# Autodesk Inventor assembly: GRUÚA
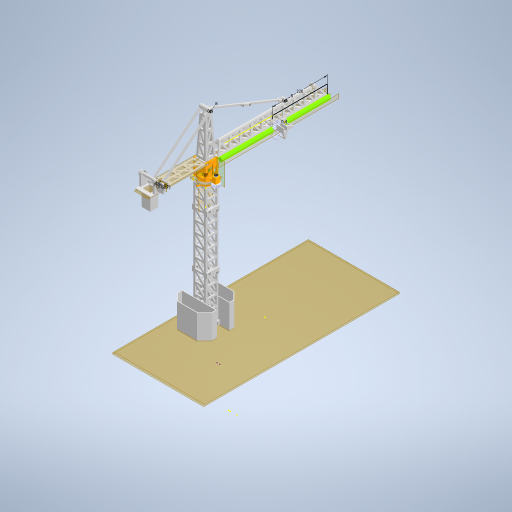
[picture p0: Inventor's stored thumbnail of the model, 512x512]
Saved by Autodesk Inventor 2023 (Build 270158000, 158)
## iProperties
Created: 2024-07-07
Part Number: GRUÚA
Document SubType Name: Assembly
Designer: Usuario
Author: Usuario
## Documents named in this file (16)
- C:\Users\Usuario\Desktop\GRUA\GRUÚA.iam
- C:\Users\Usuario\Desktop\GRUA\ALOJAMIENTO MOTOR.ipt
- C:\Users\Usuario\Desktop\GRUA\CARRIL 1.ipt
- C:\Users\Usuario\Downloads\CABLE 3_MIR.ipt
- C:\Users\Usuario\Downloads\CABLE 3_2_MIR.ipt
- C:\Users\Usuario\Downloads\CABLE 3_MIR1.ipt
- C:\Users\Usuario\Downloads\CABLE 3_2_MIR1.ipt
- C:\Users\Usuario\Downloads\CABLE 3_MIR2.ipt
- C:\Users\Usuario\Downloads\CABLE 3_2_MIR2.ipt
- C:\Users\Usuario\Desktop\GRUA\GRUA INF.ipt
- C:\Users\Usuario\Desktop\GRUA\GRÚA SUP.ipt
- C:\Users\Usuario\Documents\Inventor\Content Center Files\R2023\es-ES\ANSI B18.3.4M(1)\ANSI B18.3.4M - M4 x 0.7 x 12(2).ipt
- C:\Users\Usuario\Desktop\GRUA\Pieza26.ipt
- C:\Users\Usuario\Desktop\GRUA\Carril 1 ipt.ipt
- C:\Users\Usuario\Desktop\GRUA\Union engranaje.ipt
- C:\Users\Usuario\Desktop\GRUA\CARRIL Y RUEDAS DEFINITIVO.ipt
## Components (34 placed, 15 different names)
1. CABLE 3_MIR:1
2. CABLE 3_2_MIR:1
3. CABLE 3_MIR1:1
4. CABLE 3_2_MIR1:1
5. CABLE 3_MIR2:1
6. CABLE 3_2_MIR2:1
7. GRUA INF:1 — De rotación:6, De rotación:7, De rotación:10, De rotación:11, De rotación:12, De rotación:13, De rotación:17, De rotación:18, De rotación:19, De rotación:20, De rotación:21, De rotación:22
8. ALOJAMIENTO MOTOR:1 — De rotación:3, De rotación:26
9. GRÚA SUP:1 — De rotación:3, De rotación:5, De rotación:14, De rotación:15, De rotación:16, De rotación:23, De rotación:24, De rotación:25, Rígido:1, Coincidencia:1, Cilíndrica:1
10. CARRIL 1:1 — De rotación:5
11. Tornillo brochado de cabeza de botón hexagonal hueca - Métrico M4 x 0.7 x 12:1 — De rotación:6
12. Tornillo brochado de cabeza de botón hexagonal hueca - Métrico M4 x 0.7 x 12:2 — De rotación:12
13. Tornillo brochado de cabeza de botón hexagonal hueca - Métrico M4 x 0.7 x 12:3
14. Tornillo brochado de cabeza de botón hexagonal hueca - Métrico M4 x 0.7 x 12:4 — De rotación:10
15. Tornillo brochado de cabeza de botón hexagonal hueca - Métrico M4 x 0.7 x 12:5 — De rotación:11
16. Tornillo brochado de cabeza de botón hexagonal hueca - Métrico M4 x 0.7 x 12:6 — De rotación:13
17. Tornillo brochado de cabeza de botón hexagonal hueca - Métrico M4 x 0.7 x 12:7 — De rotación:7
18. Tornillo brochado de cabeza de botón hexagonal hueca - Métrico M4 x 0.7 x 12:8
19. Tornillo brochado de cabeza de botón hexagonal hueca - Métrico M4 x 0.7 x 12:9 — De rotación:14
20. Tornillo brochado de cabeza de botón hexagonal hueca - Métrico M4 x 0.7 x 12:10 — De rotación:16
21. Tornillo brochado de cabeza de botón hexagonal hueca - Métrico M4 x 0.7 x 12:11 — De rotación:15
22. Tornillo brochado de cabeza de botón hexagonal hueca - Métrico M4 x 0.7 x 12:12 — De rotación:17
23. Tornillo brochado de cabeza de botón hexagonal hueca - Métrico M4 x 0.7 x 12:13 — De rotación:18
24. Tornillo brochado de cabeza de botón hexagonal hueca - Métrico M4 x 0.7 x 12:14 — De rotación:19
25. Tornillo brochado de cabeza de botón hexagonal hueca - Métrico M4 x 0.7 x 12:15 — De rotación:20
26. Tornillo brochado de cabeza de botón hexagonal hueca - Métrico M4 x 0.7 x 12:16 — De rotación:21
27. Tornillo brochado de cabeza de botón hexagonal hueca - Métrico M4 x 0.7 x 12:17 — De rotación:22
28. Tornillo brochado de cabeza de botón hexagonal hueca - Métrico M4 x 0.7 x 12:18 — De rotación:23
29. Tornillo brochado de cabeza de botón hexagonal hueca - Métrico M4 x 0.7 x 12:19 — De rotación:24
30. Tornillo brochado de cabeza de botón hexagonal hueca - Métrico M4 x 0.7 x 12:20 — De rotación:25
31. Pieza26:1 — Rígido:1
32. Carril 1 ipt:1 — Coincidencia:1, Cilíndrica:1, Rígido:2
33. Union engranaje:1 — De rotación:26
34. CARRIL Y RUEDAS DEFINITIVO:1 — Rígido:2
## Relationships (25: RevoluteJoint 21, WeldJoint 2, Mate 1, CylindricalJoint 1)
- De rotación:3 [RevoluteJoint]: ALOJAMIENTO MOTOR:1 ↔ GRÚA SUP:1
- De rotación:5 [RevoluteJoint]: GRÚA SUP:1 ↔ CARRIL 1:1
- De rotación:6 [RevoluteJoint]: GRUA INF:1 ↔ Tornillo brochado de cabeza de botón hexagonal hueca - Métrico M4 x 0.7 x 12:1
- De rotación:7 [RevoluteJoint]: GRUA INF:1 ↔ Tornillo brochado de cabeza de botón hexagonal hueca - Métrico M4 x 0.7 x 12:7
- De rotación:10 [RevoluteJoint]: GRUA INF:1 ↔ Tornillo brochado de cabeza de botón hexagonal hueca - Métrico M4 x 0.7 x 12:4
- De rotación:11 [RevoluteJoint]: GRUA INF:1 ↔ Tornillo brochado de cabeza de botón hexagonal hueca - Métrico M4 x 0.7 x 12:5
- De rotación:12 [RevoluteJoint]: GRUA INF:1 ↔ Tornillo brochado de cabeza de botón hexagonal hueca - Métrico M4 x 0.7 x 12:2
- De rotación:13 [RevoluteJoint]: GRUA INF:1 ↔ Tornillo brochado de cabeza de botón hexagonal hueca - Métrico M4 x 0.7 x 12:6
- De rotación:14 [RevoluteJoint]: GRÚA SUP:1 ↔ Tornillo brochado de cabeza de botón hexagonal hueca - Métrico M4 x 0.7 x 12:9
- De rotación:15 [RevoluteJoint]: GRÚA SUP:1 ↔ Tornillo brochado de cabeza de botón hexagonal hueca - Métrico M4 x 0.7 x 12:11
- De rotación:16 [RevoluteJoint]: GRÚA SUP:1 ↔ Tornillo brochado de cabeza de botón hexagonal hueca - Métrico M4 x 0.7 x 12:10
- De rotación:17 [RevoluteJoint]: GRUA INF:1 ↔ Tornillo brochado de cabeza de botón hexagonal hueca - Métrico M4 x 0.7 x 12:12
- De rotación:18 [RevoluteJoint]: GRUA INF:1 ↔ Tornillo brochado de cabeza de botón hexagonal hueca - Métrico M4 x 0.7 x 12:13
- De rotación:19 [RevoluteJoint]: GRUA INF:1 ↔ Tornillo brochado de cabeza de botón hexagonal hueca - Métrico M4 x 0.7 x 12:14
- De rotación:20 [RevoluteJoint]: GRUA INF:1 ↔ Tornillo brochado de cabeza de botón hexagonal hueca - Métrico M4 x 0.7 x 12:15
- De rotación:21 [RevoluteJoint]: GRUA INF:1 ↔ Tornillo brochado de cabeza de botón hexagonal hueca - Métrico M4 x 0.7 x 12:16
- De rotación:22 [RevoluteJoint]: GRUA INF:1 ↔ Tornillo brochado de cabeza de botón hexagonal hueca - Métrico M4 x 0.7 x 12:17
- De rotación:23 [RevoluteJoint]: GRÚA SUP:1 ↔ Tornillo brochado de cabeza de botón hexagonal hueca - Métrico M4 x 0.7 x 12:18
- De rotación:24 [RevoluteJoint]: GRÚA SUP:1 ↔ Tornillo brochado de cabeza de botón hexagonal hueca - Métrico M4 x 0.7 x 12:19
- De rotación:25 [RevoluteJoint]: GRÚA SUP:1 ↔ Tornillo brochado de cabeza de botón hexagonal hueca - Métrico M4 x 0.7 x 12:20
- Rígido:1 [WeldJoint]: GRÚA SUP:1 ↔ Pieza26:1
- Coincidencia:1 [Mate]: GRÚA SUP:1 ↔ Carril 1 ipt:1
- Cilíndrica:1 [CylindricalJoint]: GRÚA SUP:1 ↔ Carril 1 ipt:1
- De rotación:26 [RevoluteJoint]: ALOJAMIENTO MOTOR:1 ↔ Union engranaje:1
- Rígido:2 [WeldJoint]: Carril 1 ipt:1 ↔ CARRIL Y RUEDAS DEFINITIVO:1
